# Autodesk Inventor assembly: ASSEMBLY_Main
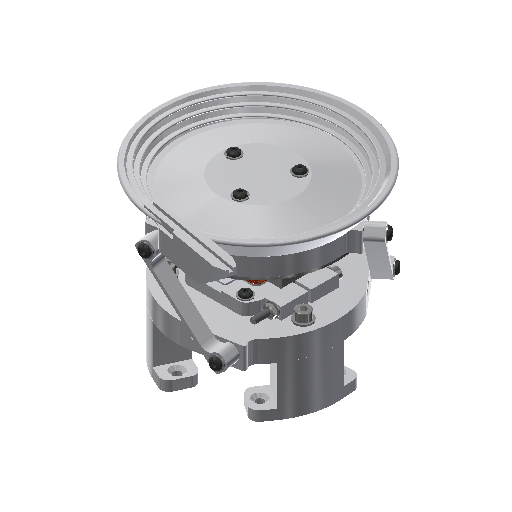
[picture p0: Inventor's stored thumbnail of the model, 512x512]
Saved by Autodesk Inventor 2025 (Build 290162010, 162A)
## iProperties
Created: 2018-05-26
Part Number: ASSEMBLY_Main
Document SubType Name: Assembly
Designer: Andrzej
Author: Andrzej
## Documents named in this file (15)
- D:\_ANDRZEJ_LACZEWSKI\_OTHER\MLTDIS - SMD parts bowl feeder prototype\MCAD\1_REV1\ASSEMBLY_MAIN_REVA\ASSEMBLY_Main.iam
- D:\_ANDRZEJ_LACZEWSKI\_OTHER\MLTDIS - SMD parts bowl feeder prototype\MCAD\1_REV1\ASSEMBLY_MAIN_REVA\3DP_ABS_Bowl_Feeder_Base_Plate.ipt
- D:\_ANDRZEJ_LACZEWSKI\_OTHER\MLTDIS - SMD parts bowl feeder prototype\MCAD\1_REV1\ASSEMBLY_MAIN_REVA\ASSEMBLY_Electromagnet.iam
- D:\_ANDRZEJ_LACZEWSKI\_OTHER\MLTDIS - SMD parts bowl feeder prototype\MCAD\1_REV1\ASSEMBLY_MAIN_REVA\3DP_ABS_Bowl_For_1206_SMD_Components.ipt
- D:\_ANDRZEJ_LACZEWSKI\_OTHER\MLTDIS - SMD parts bowl feeder prototype\MCAD\1_REV1\ASSEMBLY_MAIN_REVA\3DP_ABS_Bowl_Springs_Mount_Plate.ipt
- D:\_ANDRZEJ_LACZEWSKI\_OTHER\MLTDIS - SMD parts bowl feeder prototype\MCAD\1_REV1\ASSEMBLY_MAIN_REVA\3DP_ABS_Bowl_Spring.ipt
- D:\_ANDRZEJ_LACZEWSKI\_OTHER\MLTDIS - SMD parts bowl feeder prototype\MCAD\1_REV1\ASSEMBLY_MAIN_REVA\CNCM_STEEL_Bowl_Electromagnet_Plate.ipt
- D:\_ANDRZEJ_LACZEWSKI\_OTHER\MLTDIS - SMD parts bowl feeder prototype\MCAD\1_REV1\ASSEMBLY_MAIN_REVA\3DP_ABS_Bowl_Feeder_Standoff.ipt
- D:\_ANDRZEJ_LACZEWSKI\_OTHER\MLTDIS - SMD parts bowl feeder prototype\MCAD\1_REV1\__CONTENT_CENTER_PARTS\en-US\DIN 125-2  A\DIN 125-2 - A 3,2A.ipt
- D:\_ANDRZEJ_LACZEWSKI\_OTHER\MLTDIS - SMD parts bowl feeder prototype\MCAD\1_REV1\__CONTENT_CENTER_PARTS\en-US\ISO 7380-1\ISO 7380-1 - M3 x 20.ipt
- D:\_ANDRZEJ_LACZEWSKI\_OTHER\MLTDIS - SMD parts bowl feeder prototype\MCAD\1_REV1\__CONTENT_CENTER_PARTS\en-US\DIN 934\DIN 934 - M3 x 0,5.ipt
- D:\_ANDRZEJ_LACZEWSKI\_OTHER\MLTDIS - SMD parts bowl feeder prototype\MCAD\1_REV1\__CONTENT_CENTER_PARTS\en-US\DIN 125-2  A\DIN 125-2 - A 4,3A.ipt
- D:\_ANDRZEJ_LACZEWSKI\_OTHER\MLTDIS - SMD parts bowl feeder prototype\MCAD\1_REV1\__CONTENT_CENTER_PARTS\en-US\DIN 912\DIN 912 - M4 x 0,7 x 25 x 23,25.ipt
- D:\_ANDRZEJ_LACZEWSKI\_OTHER\MLTDIS - SMD parts bowl feeder prototype\MCAD\1_REV1\__CONTENT_CENTER_PARTS\en-US\ISO 7380-1\ISO 7380-1 - M3 x 12.ipt
- D:\_ANDRZEJ_LACZEWSKI\_OTHER\MLTDIS - SMD parts bowl feeder prototype\MCAD\1_REV1\__CONTENT_CENTER_PARTS\en-US\ISO 7380-1\ISO 7380-1 - M3 x 8.ipt
## Components (63 placed, 14 different names)
1. 3DP_ABS_Bowl_Feeder_Base_Plate:1 — Mate:1, Mate:3, Mate:4, Mate:7, Flush:1, Mate:8, Mate:9, Mate:17, Mate:18, Mate:19, Mate:20, Mate:21, Mate:22, Mate:23, Mate:24, Mate:25, Mate:35, Mate:37, Mate:39, Mate:41, Mate:47, Mate:48, Mate:49, Mate:50, Mate:51, Mate:52
2. ASSEMBLY_Electromagnet:1 [sub-assembly] — Mate:1, Mate:3, Mate:4, Mate:26, Mate:27, Mate:28, Mate:29, Mate:30, Mate:31, Mate:32, Mate:33, Mate:34, Mate:36, Mate:38, Mate:40
3. 3DP_ABS_Bowl_Springs_Mount_Plate:1 — Mate:7, Flush:1, Mate:10, Mate:11, Mate:12, Mate:13, Mate:14, Mate:15, Mate:16, Mate:46, Mate:65, Mate:67
4. 3DP_ABS_Bowl_For_1206_SMD_Components:1 — Mate:11, Mate:12, Mate:15, Mate:53, Mate:54, Mate:55, Mate:56, Mate:57, Mate:58
5. CNCM_STEEL_Bowl_Electromagnet_Plate:1 — Mate:13, Mate:14, Mate:16, Mate:59, Mate:60, Mate:61, Mate:62, Mate:63, Mate:64, Mate:66, Mate:68, Mate:69, Mate:70
6. 3DP_ABS_Bowl_Feeder_Standoff:1 — Mate:17, Mate:20, Mate:23
7. 3DP_ABS_Bowl_Feeder_Standoff:2 — Mate:18, Mate:22, Mate:25
8. 3DP_ABS_Bowl_Feeder_Standoff:3 — Mate:19, Mate:21, Mate:24
9. ISO 7380-1 M3 x 8:6 — Insert:22
10. ISO 7380-1 M3 x 8:5 — Insert:21
11. ISO 7380-1 M3 x 8:4 — Insert:20
12. ISO 7380-1 M3 x 8:3 — Insert:19
13. ISO 7380-1 M3 x 8:2 — Insert:18
14. DIN 125-2 A A 3,2:23 — Mate:69, Mate:70, Insert:22
15. DIN 125-2 A A 3,2:22 — Mate:67, Mate:68, Insert:21
16. DIN 125-2 A A 3,2:21 — Mate:65, Mate:66, Insert:20
17. DIN 125-2 A A 3,2:20 — Mate:63, Mate:64, Insert:19
18. DIN 125-2 A A 3,2:19 — Mate:61, Mate:62, Insert:18
19. ISO 7380-1 M3 x 8:1 — Insert:17
20. DIN 125-2 A A 3,2:18 — Mate:59, Mate:60, Insert:17
21. ISO 7380-1 M3 x 12:3 — Insert:16
22. ISO 7380-1 M3 x 12:2 — Insert:15
23. DIN 125-2 A A 3,2:17 — Mate:57, Mate:58, Insert:16
24. DIN 125-2 A A 3,2:16 — Mate:55, Mate:56, Insert:15
25. ISO 7380-1 M3 x 12:1 — Insert:14
26. DIN 125-2 A A 3,2:15 — Mate:53, Mate:54, Insert:14
27. DIN 912 - replaced by DIN EN ISO 4762 M4 x 25:3 — Insert:13
28. DIN 912 - replaced by DIN EN ISO 4762 M4 x 25:2 — Insert:12
29. DIN 125-2 A A 4,3:3 — Mate:51, Mate:52, Insert:13
30. DIN 125-2 A A 4,3:2 — Mate:49, Mate:50, Insert:12
31. DIN 912 - replaced by DIN EN ISO 4762 M4 x 25:1 — Insert:11
32. DIN 125-2 A A 4,3:1 — Mate:47, Mate:48, Insert:11
33. DIN 934 - replaced by DIN EN 24032/28673/28674 M3:4 — Insert:8
34. DIN 934 - replaced by DIN EN 24032/28673/28674 M3:3 — Insert:7
35. DIN 934 - replaced by DIN EN 24032/28673/28674 M3:2 — Insert:6
36. DIN 125-2 A A 3,2:8 — Mate:40, Mate:41, Insert:8
37. DIN 125-2 A A 3,2:7 — Mate:38, Mate:39, Insert:7
38. DIN 125-2 A A 3,2:6 — Mate:36, Mate:37, Insert:6
39. ISO 7380-1 M3 x 20:4 — Insert:4
40. ISO 7380-1 M3 x 20:3 — Insert:3
41. ISO 7380-1 M3 x 20:2 — Insert:2
42. DIN 125-2 A A 3,2:5 — Mate:32, Mate:33, Insert:4
43. DIN 125-2 A A 3,2:4 — Mate:30, Mate:31, Insert:3
44. DIN 125-2 A A 3,2:3 — Mate:28, Mate:29, Insert:2
45. DIN 934 - replaced by DIN EN 24032/28673/28674 M3:1 — Insert:5
46. DIN 125-2 A A 3,2:2 — Mate:34, Mate:35, Insert:5
47. ISO 7380-1 M3 x 20:1 — Insert:1
48. DIN 125-2 A A 3,2:1 — Mate:26, Mate:27, Insert:1
49. 3DP_ABS_Bowl_Spring:1 — Mate:8, Mate:9, Mate:10
50. 3DP_ABS_Bowl_Spring:2 — Mate:42, Mate:43, Mate:44, Mate:45
51. 3DP_ABS_Bowl_Spring:3
52. ISO 7380-1 M3 x 20:5 — Insert:9
53. DIN 125-2 A A 3,2:9 — Mate:42, Mate:43, Insert:9
54. ISO 7380-1 M3 x 20:6 — Insert:10
55. DIN 125-2 A A 3,2:10 — Mate:44, Mate:45, Insert:10
56. ISO 7380-1 M3 x 20:7
57. DIN 125-2 A A 3,2:11
58. ISO 7380-1 M3 x 20:8
59. DIN 125-2 A A 3,2:12
60. ISO 7380-1 M3 x 20:9
61. DIN 125-2 A A 3,2:13
62. ISO 7380-1 M3 x 20:10
63. DIN 125-2 A A 3,2:14
## Component patterns: (3 elements, first: 3DP_ABS_Bowl_Spring:1), (3 elements, first: ISO 7380-1 M3 x 20:5 + DIN 125-2 A A 3,2:9 + ISO 7380-1 M3 x 20:6 + DIN 125-2 A A 3,2:10)
## Relationships (90: Mate 67, Insert 22, Flush 1)
- Mate:1: 3DP_ABS_Bowl_Feeder_Base_Plate:1 ↔ ASSEMBLY_Electromagnet:1
- Mate:3: 3DP_ABS_Bowl_Feeder_Base_Plate:1 ↔ ASSEMBLY_Electromagnet:1
- Mate:4: 3DP_ABS_Bowl_Feeder_Base_Plate:1 ↔ ASSEMBLY_Electromagnet:1
- Mate:7: 3DP_ABS_Bowl_Feeder_Base_Plate:1 ↔ 3DP_ABS_Bowl_Springs_Mount_Plate:1
- Flush:1: 3DP_ABS_Bowl_Feeder_Base_Plate:1 ↔ 3DP_ABS_Bowl_Springs_Mount_Plate:1
- Mate:8: 3DP_ABS_Bowl_Feeder_Base_Plate:1 ↔ 3DP_ABS_Bowl_Spring:1
- Mate:9: 3DP_ABS_Bowl_Feeder_Base_Plate:1 ↔ 3DP_ABS_Bowl_Spring:1
- Mate:10: 3DP_ABS_Bowl_Springs_Mount_Plate:1 ↔ 3DP_ABS_Bowl_Spring:1
- Mate:11: 3DP_ABS_Bowl_Springs_Mount_Plate:1 ↔ 3DP_ABS_Bowl_For_1206_SMD_Components:1
- Mate:12: 3DP_ABS_Bowl_Springs_Mount_Plate:1 ↔ 3DP_ABS_Bowl_For_1206_SMD_Components:1
- Mate:13: 3DP_ABS_Bowl_Springs_Mount_Plate:1 ↔ CNCM_STEEL_Bowl_Electromagnet_Plate:1
- Mate:14: 3DP_ABS_Bowl_Springs_Mount_Plate:1 ↔ CNCM_STEEL_Bowl_Electromagnet_Plate:1
- Mate:15: 3DP_ABS_Bowl_Springs_Mount_Plate:1 ↔ 3DP_ABS_Bowl_For_1206_SMD_Components:1
- Mate:16: 3DP_ABS_Bowl_Springs_Mount_Plate:1 ↔ CNCM_STEEL_Bowl_Electromagnet_Plate:1
- Mate:17: 3DP_ABS_Bowl_Feeder_Base_Plate:1 ↔ 3DP_ABS_Bowl_Feeder_Standoff:1
- Mate:18: 3DP_ABS_Bowl_Feeder_Base_Plate:1 ↔ 3DP_ABS_Bowl_Feeder_Standoff:2
- Mate:19: 3DP_ABS_Bowl_Feeder_Base_Plate:1 ↔ 3DP_ABS_Bowl_Feeder_Standoff:3
- Mate:20: 3DP_ABS_Bowl_Feeder_Base_Plate:1 ↔ 3DP_ABS_Bowl_Feeder_Standoff:1
- Mate:21: 3DP_ABS_Bowl_Feeder_Base_Plate:1 ↔ 3DP_ABS_Bowl_Feeder_Standoff:3
- Mate:22: 3DP_ABS_Bowl_Feeder_Base_Plate:1 ↔ 3DP_ABS_Bowl_Feeder_Standoff:2
- Mate:23: 3DP_ABS_Bowl_Feeder_Base_Plate:1 ↔ 3DP_ABS_Bowl_Feeder_Standoff:1
- Mate:24: 3DP_ABS_Bowl_Feeder_Base_Plate:1 ↔ 3DP_ABS_Bowl_Feeder_Standoff:3
- Mate:25: 3DP_ABS_Bowl_Feeder_Base_Plate:1 ↔ 3DP_ABS_Bowl_Feeder_Standoff:2
- Mate:26: ASSEMBLY_Electromagnet:1 ↔ DIN 125-2 A A 3,2:1
- Mate:27: ASSEMBLY_Electromagnet:1 ↔ DIN 125-2 A A 3,2:1
- Mate:28: ASSEMBLY_Electromagnet:1 ↔ DIN 125-2 A A 3,2:3
- Mate:29: ASSEMBLY_Electromagnet:1 ↔ DIN 125-2 A A 3,2:3
- Mate:30: ASSEMBLY_Electromagnet:1 ↔ DIN 125-2 A A 3,2:4
- Mate:31: ASSEMBLY_Electromagnet:1 ↔ DIN 125-2 A A 3,2:4
- Mate:32: ASSEMBLY_Electromagnet:1 ↔ DIN 125-2 A A 3,2:5
- Mate:33: ASSEMBLY_Electromagnet:1 ↔ DIN 125-2 A A 3,2:5
- Insert:1: ISO 7380-1 M3 x 20:1 ↔ DIN 125-2 A A 3,2:1
- Insert:2: ISO 7380-1 M3 x 20:2 ↔ DIN 125-2 A A 3,2:3
- Insert:3: ISO 7380-1 M3 x 20:3 ↔ DIN 125-2 A A 3,2:4
- Insert:4: ISO 7380-1 M3 x 20:4 ↔ DIN 125-2 A A 3,2:5
- Mate:34: ASSEMBLY_Electromagnet:1 ↔ DIN 125-2 A A 3,2:2
- Mate:35: 3DP_ABS_Bowl_Feeder_Base_Plate:1 ↔ DIN 125-2 A A 3,2:2
- Mate:36: ASSEMBLY_Electromagnet:1 ↔ DIN 125-2 A A 3,2:6
- Mate:37: 3DP_ABS_Bowl_Feeder_Base_Plate:1 ↔ DIN 125-2 A A 3,2:6
- Mate:38: ASSEMBLY_Electromagnet:1 ↔ DIN 125-2 A A 3,2:7
- Mate:39: 3DP_ABS_Bowl_Feeder_Base_Plate:1 ↔ DIN 125-2 A A 3,2:7
- Mate:40: ASSEMBLY_Electromagnet:1 ↔ DIN 125-2 A A 3,2:8
- Mate:41: 3DP_ABS_Bowl_Feeder_Base_Plate:1 ↔ DIN 125-2 A A 3,2:8
- Insert:5: DIN 934 - replaced by DIN EN 24032/28673/28674 M3:1 ↔ DIN 125-2 A A 3,2:2
- Insert:6: DIN 934 - replaced by DIN EN 24032/28673/28674 M3:2 ↔ DIN 125-2 A A 3,2:6
- Insert:7: DIN 934 - replaced by DIN EN 24032/28673/28674 M3:3 ↔ DIN 125-2 A A 3,2:7
- Insert:8: DIN 934 - replaced by DIN EN 24032/28673/28674 M3:4 ↔ DIN 125-2 A A 3,2:8
- Mate:42: 3DP_ABS_Bowl_Spring:2 ↔ DIN 125-2 A A 3,2:9
- Mate:43: 3DP_ABS_Bowl_Spring:2 ↔ DIN 125-2 A A 3,2:9
- Mate:44: 3DP_ABS_Bowl_Spring:2 ↔ DIN 125-2 A A 3,2:10
- Mate:45: 3DP_ABS_Bowl_Spring:2 ↔ DIN 125-2 A A 3,2:10
- Insert:9: ISO 7380-1 M3 x 20:5 ↔ DIN 125-2 A A 3,2:9
- Insert:10: ISO 7380-1 M3 x 20:6 ↔ DIN 125-2 A A 3,2:10
- Mate:46: 3DP_ABS_Bowl_Springs_Mount_Plate:1
- Mate:47: 3DP_ABS_Bowl_Feeder_Base_Plate:1 ↔ DIN 125-2 A A 4,3:1
- Mate:48: 3DP_ABS_Bowl_Feeder_Base_Plate:1 ↔ DIN 125-2 A A 4,3:1
- Mate:49: 3DP_ABS_Bowl_Feeder_Base_Plate:1 ↔ DIN 125-2 A A 4,3:2
- Mate:50: 3DP_ABS_Bowl_Feeder_Base_Plate:1 ↔ DIN 125-2 A A 4,3:2
- Mate:51: 3DP_ABS_Bowl_Feeder_Base_Plate:1 ↔ DIN 125-2 A A 4,3:3
- Mate:52: 3DP_ABS_Bowl_Feeder_Base_Plate:1 ↔ DIN 125-2 A A 4,3:3
- Insert:11: DIN 912 - replaced by DIN EN ISO 4762 M4 x 25:1 ↔ DIN 125-2 A A 4,3:1
- Insert:12: DIN 912 - replaced by DIN EN ISO 4762 M4 x 25:2 ↔ DIN 125-2 A A 4,3:2
- Insert:13: DIN 912 - replaced by DIN EN ISO 4762 M4 x 25:3 ↔ DIN 125-2 A A 4,3:3
- Mate:53: 3DP_ABS_Bowl_For_1206_SMD_Components:1 ↔ DIN 125-2 A A 3,2:15
- Mate:54: 3DP_ABS_Bowl_For_1206_SMD_Components:1 ↔ DIN 125-2 A A 3,2:15
- Mate:55: 3DP_ABS_Bowl_For_1206_SMD_Components:1 ↔ DIN 125-2 A A 3,2:16
- Mate:56: 3DP_ABS_Bowl_For_1206_SMD_Components:1 ↔ DIN 125-2 A A 3,2:16
- Mate:57: 3DP_ABS_Bowl_For_1206_SMD_Components:1 ↔ DIN 125-2 A A 3,2:17
- Mate:58: 3DP_ABS_Bowl_For_1206_SMD_Components:1 ↔ DIN 125-2 A A 3,2:17
- Insert:14: ISO 7380-1 M3 x 12:1 ↔ DIN 125-2 A A 3,2:15
- Insert:15: ISO 7380-1 M3 x 12:2 ↔ DIN 125-2 A A 3,2:16
- Insert:16: ISO 7380-1 M3 x 12:3 ↔ DIN 125-2 A A 3,2:17
- Mate:59: CNCM_STEEL_Bowl_Electromagnet_Plate:1 ↔ DIN 125-2 A A 3,2:18
- Mate:60: CNCM_STEEL_Bowl_Electromagnet_Plate:1 ↔ DIN 125-2 A A 3,2:18
- Mate:61: CNCM_STEEL_Bowl_Electromagnet_Plate:1 ↔ DIN 125-2 A A 3,2:19
- Mate:62: CNCM_STEEL_Bowl_Electromagnet_Plate:1 ↔ DIN 125-2 A A 3,2:19
- Mate:63: CNCM_STEEL_Bowl_Electromagnet_Plate:1 ↔ DIN 125-2 A A 3,2:20
- Mate:64: CNCM_STEEL_Bowl_Electromagnet_Plate:1 ↔ DIN 125-2 A A 3,2:20
- Mate:65: 3DP_ABS_Bowl_Springs_Mount_Plate:1 ↔ DIN 125-2 A A 3,2:21
- Mate:66: CNCM_STEEL_Bowl_Electromagnet_Plate:1 ↔ DIN 125-2 A A 3,2:21
- Mate:67: 3DP_ABS_Bowl_Springs_Mount_Plate:1 ↔ DIN 125-2 A A 3,2:22
- Mate:68: CNCM_STEEL_Bowl_Electromagnet_Plate:1 ↔ DIN 125-2 A A 3,2:22
- Mate:69: CNCM_STEEL_Bowl_Electromagnet_Plate:1 ↔ DIN 125-2 A A 3,2:23
- Mate:70: CNCM_STEEL_Bowl_Electromagnet_Plate:1 ↔ DIN 125-2 A A 3,2:23
- Insert:17: ISO 7380-1 M3 x 8:1 ↔ DIN 125-2 A A 3,2:18
- Insert:18: ISO 7380-1 M3 x 8:2 ↔ DIN 125-2 A A 3,2:19
- Insert:19: ISO 7380-1 M3 x 8:3 ↔ DIN 125-2 A A 3,2:20
- Insert:20: ISO 7380-1 M3 x 8:4 ↔ DIN 125-2 A A 3,2:21
- Insert:21: ISO 7380-1 M3 x 8:5 ↔ DIN 125-2 A A 3,2:22
- Insert:22: ISO 7380-1 M3 x 8:6 ↔ DIN 125-2 A A 3,2:23
